# Autodesk Inventor assembly: 組合2
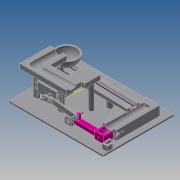
[picture p0: Inventor's stored thumbnail of the model, 180x180]
Saved by Autodesk Inventor 2015 (Build 190159000, 159)
## iProperties
Created: 2017-12-26
Part Number: 組合2
Document SubType Name: Assembly
Designer: user
Author: user
## Documents named in this file (11)
- C:\Users\user\Desktop\電腦輔助設計\組合2.iam
- C:\Users\user\Desktop\電腦輔助設計\01底板.ipt
- C:\Users\user\Desktop\電腦輔助設計\02連桿25.ipt
- C:\Users\user\Desktop\電腦輔助設計\03連桿15.ipt
- C:\Users\user\Desktop\電腦輔助設計\馬達.ipt
- C:\Users\user\Desktop\電腦輔助設計\連趕2.ipt
- C:\Users\user\Desktop\電腦輔助設計\槓桿.ipt
- C:\Users\user\Desktop\電腦輔助設計\個人\滑軌.ipt
- C:\Users\user\Desktop\電腦輔助設計\個人\滑軌3.ipt
- C:\Users\user\Desktop\電腦輔助設計\長銷.ipt
- C:\Users\user\Desktop\電腦輔助設計\銷.ipt
## Components (17 placed, 10 different names)
1. 01底板:1 — 插入:1, 貼合:1, 插入:4, 貼合:4, 角度:1, 插入:5, 貼合:6, 貼合:7, 貼合:8, 齊平:1, 插入:6, 貼合:9, 貼合:10, 貼合:11, 貼合:15
2. 02連桿25:1 — 插入:3, 貼合:3
3. 03連桿15:1 — 貼合:2, 插入:2, 插入:3, 角度:1, 貼合:12, 貼合:13
4. 馬達:1 — 插入:1, 貼合:1, 貼合:2
5. 連趕2:1 — 插入:4, 貼合:5
6. 02連桿25:2 — 插入:2, 貼合:3, 貼合:4, 貼合:5, 貼合:14
7. 槓桿:2 — 插入:5
8. 滑軌:1 — 貼合:6
9. 滑軌3:1 — 貼合:7, 貼合:8, 齊平:1
10. 長銷:1 — 插入:6
11. 銷:1 — 貼合:10
12. 銷:2 — 貼合:11
13. 銷:4 — 貼合:9
14. 銷:5 — 貼合:15
15. 銷:6 — 貼合:12
16. 銷:7 — 貼合:13
17. 長銷:2 — 貼合:14
## Relationships (23: Mate 15, Insert 6, Angle 1, Flush 1)
- 插入:1 [Insert]: 01底板:1 ↔ 馬達:1
- 貼合:1 [Mate]: 01底板:1 ↔ 馬達:1
- 貼合:2 [Mate]: 03連桿15:1 ↔ 馬達:1
- 插入:2 [Insert]: 03連桿15:1 ↔ 02連桿25:2
- 插入:3 [Insert]: 02連桿25:1 ↔ 03連桿15:1
- 貼合:3 [Mate]: 02連桿25:1 ↔ 02連桿25:2
- 插入:4 [Insert]: 01底板:1 ↔ 連趕2:1
- 貼合:4 [Mate]: 01底板:1 ↔ 02連桿25:2
- 貼合:5 [Mate]: 連趕2:1 ↔ 02連桿25:2
- 角度:1 [Angle] (0 deg): 01底板:1 ↔ 03連桿15:1
- 插入:5 [Insert] (-10 mm): 01底板:1 ↔ 槓桿:2
- 貼合:6 [Mate]: 01底板:1 ↔ 滑軌:1
- 貼合:7 [Mate]: 01底板:1 ↔ 滑軌3:1
- 貼合:8 [Mate]: 01底板:1 ↔ 滑軌3:1
- 齊平:1 [Flush] (-42 mm): 01底板:1 ↔ 滑軌3:1
- 插入:6 [Insert]: 01底板:1 ↔ 長銷:1
- 貼合:9 [Mate]: 01底板:1 ↔ 銷:4
- 貼合:10 [Mate]: 01底板:1 ↔ 銷:1
- 貼合:11 [Mate]: 01底板:1 ↔ 銷:2
- 貼合:12 [Mate]: 03連桿15:1 ↔ 銷:6
- 貼合:13 [Mate]: 03連桿15:1 ↔ 銷:7
- 貼合:14 [Mate]: 02連桿25:2 ↔ 長銷:2
- 貼合:15 [Mate]: 01底板:1 ↔ 銷:5
